(part 1 of 4)
# Autodesk Inventor assembly: FRC Fixed Field 2018_sldasm
Saved by Autodesk Inventor 2016 SP2 (Build 200236200, 236)
## iProperties
Created: 2018-01-13
Part Number: FRC Fixed Field 2018_sldasm
Document SubType Name: Assembly
Designer: CAD
Author: CAD
## Documents named in this file (943)
- C:\Users\CAD\Documents\GitHub\FIRST-ROBOTICS-2018-5436-CAD\Field\FIRST Power Up Field CAD\FRC Fixed Field 2018_sldasm.iam
- C:\Users\CAD\Documents\GitHub\FIRST-ROBOTICS-2018-5436-CAD\Field\FIRST Power Up Field CAD\Body_525_sldprt.ipt
- C:\Users\CAD\Documents\GitHub\FIRST-ROBOTICS-2018-5436-CAD\Field\FIRST Power Up Field CAD\Body_526_sldprt.ipt
- C:\Users\CAD\Documents\GitHub\FIRST-ROBOTICS-2018-5436-CAD\Field\FIRST Power Up Field CAD\Body_527_sldprt.ipt
- C:\Users\CAD\Documents\GitHub\FIRST-ROBOTICS-2018-5436-CAD\Field\FIRST Power Up Field CAD\Body_528_sldprt.ipt
- C:\Users\CAD\Documents\GitHub\FIRST-ROBOTICS-2018-5436-CAD\Field\FIRST Power Up Field CAD\Body_529_sldprt.ipt
- C:\Users\CAD\Documents\GitHub\FIRST-ROBOTICS-2018-5436-CAD\Field\FIRST Power Up Field CAD\Body_530_sldprt.ipt
- C:\Users\CAD\Documents\GitHub\FIRST-ROBOTICS-2018-5436-CAD\Field\FIRST Power Up Field CAD\Body_531_sldprt.ipt
- C:\Users\CAD\Documents\GitHub\FIRST-ROBOTICS-2018-5436-CAD\Field\FIRST Power Up Field CAD\Body_532_sldprt.ipt
- C:\Users\CAD\Documents\GitHub\FIRST-ROBOTICS-2018-5436-CAD\Field\FIRST Power Up Field CAD\Body_533_sldprt.ipt
- C:\Users\CAD\Documents\GitHub\FIRST-ROBOTICS-2018-5436-CAD\Field\FIRST Power Up Field CAD\Body_534_sldprt.ipt
- C:\Users\CAD\Documents\GitHub\FIRST-ROBOTICS-2018-5436-CAD\Field\FIRST Power Up Field CAD\Body_535_sldprt.ipt
- C:\Users\CAD\Documents\GitHub\FIRST-ROBOTICS-2018-5436-CAD\Field\FIRST Power Up Field CAD\Body_536_sldprt.ipt
- C:\Users\CAD\Documents\GitHub\FIRST-ROBOTICS-2018-5436-CAD\Field\FIRST Power Up Field CAD\Body_537_sldprt.ipt
- C:\Users\CAD\Documents\GitHub\FIRST-ROBOTICS-2018-5436-CAD\Field\FIRST Power Up Field CAD\Body_538_sldprt.ipt
- C:\Users\CAD\Documents\GitHub\FIRST-ROBOTICS-2018-5436-CAD\Field\FIRST Power Up Field CAD\Body_539_sldprt.ipt
- C:\Users\CAD\Documents\GitHub\FIRST-ROBOTICS-2018-5436-CAD\Field\FIRST Power Up Field CAD\Body_540_sldprt.ipt
- C:\Users\CAD\Documents\GitHub\FIRST-ROBOTICS-2018-5436-CAD\Field\FIRST Power Up Field CAD\Body_541_sldprt.ipt
- C:\Users\CAD\Documents\GitHub\FIRST-ROBOTICS-2018-5436-CAD\Field\FIRST Power Up Field CAD\Body_542_sldprt.ipt
- C:\Users\CAD\Documents\GitHub\FIRST-ROBOTICS-2018-5436-CAD\Field\FIRST Power Up Field CAD\Body_543_sldprt.ipt
- C:\Users\CAD\Documents\GitHub\FIRST-ROBOTICS-2018-5436-CAD\Field\FIRST Power Up Field CAD\Body_544_sldprt.ipt
- C:\Users\CAD\Documents\GitHub\FIRST-ROBOTICS-2018-5436-CAD\Field\FIRST Power Up Field CAD\Body_545_sldprt.ipt
- C:\Users\CAD\Documents\GitHub\FIRST-ROBOTICS-2018-5436-CAD\Field\FIRST Power Up Field CAD\Body_546_sldprt.ipt
- C:\Users\CAD\Documents\GitHub\FIRST-ROBOTICS-2018-5436-CAD\Field\FIRST Power Up Field CAD\Body_547_sldprt.ipt
- C:\Users\CAD\Documents\GitHub\FIRST-ROBOTICS-2018-5436-CAD\Field\FIRST Power Up Field CAD\Body_548_sldprt.ipt
- C:\Users\CAD\Documents\GitHub\FIRST-ROBOTICS-2018-5436-CAD\Field\FIRST Power Up Field CAD\Body_549_sldprt.ipt
- C:\Users\CAD\Documents\GitHub\FIRST-ROBOTICS-2018-5436-CAD\Field\FIRST Power Up Field CAD\Body_550_sldprt.ipt
- C:\Users\CAD\Documents\GitHub\FIRST-ROBOTICS-2018-5436-CAD\Field\FIRST Power Up Field CAD\Body_551_sldprt.ipt
- C:\Users\CAD\Documents\GitHub\FIRST-ROBOTICS-2018-5436-CAD\Field\FIRST Power Up Field CAD\Body_552_sldprt.ipt
- C:\Users\CAD\Documents\GitHub\FIRST-ROBOTICS-2018-5436-CAD\Field\FIRST Power Up Field CAD\Body_553_sldprt.ipt
- C:\Users\CAD\Documents\GitHub\FIRST-ROBOTICS-2018-5436-CAD\Field\FIRST Power Up Field CAD\Body_554_sldprt.ipt
- C:\Users\CAD\Documents\GitHub\FIRST-ROBOTICS-2018-5436-CAD\Field\FIRST Power Up Field CAD\Body_555_sldprt.ipt
- C:\Users\CAD\Documents\GitHub\FIRST-ROBOTICS-2018-5436-CAD\Field\FIRST Power Up Field CAD\Body_556_sldprt.ipt
- C:\Users\CAD\Documents\GitHub\FIRST-ROBOTICS-2018-5436-CAD\Field\FIRST Power Up Field CAD\Body_557_sldprt.ipt
- C:\Users\CAD\Documents\GitHub\FIRST-ROBOTICS-2018-5436-CAD\Field\FIRST Power Up Field CAD\Body_558_sldprt.ipt
- C:\Users\CAD\Documents\GitHub\FIRST-ROBOTICS-2018-5436-CAD\Field\FIRST Power Up Field CAD\Body_559_sldprt.ipt
- C:\Users\CAD\Documents\GitHub\FIRST-ROBOTICS-2018-5436-CAD\Field\FIRST Power Up Field CAD\Body_560_sldprt.ipt
- C:\Users\CAD\Documents\GitHub\FIRST-ROBOTICS-2018-5436-CAD\Field\FIRST Power Up Field CAD\Body_561_sldprt.ipt
- C:\Users\CAD\Documents\GitHub\FIRST-ROBOTICS-2018-5436-CAD\Field\FIRST Power Up Field CAD\Body_562_sldprt.ipt
- C:\Users\CAD\Documents\GitHub\FIRST-ROBOTICS-2018-5436-CAD\Field\FIRST Power Up Field CAD\Body_563_sldprt.ipt
- C:\Users\CAD\Documents\GitHub\FIRST-ROBOTICS-2018-5436-CAD\Field\FIRST Power Up Field CAD\Body_564_sldprt.ipt
- C:\Users\CAD\Documents\GitHub\FIRST-ROBOTICS-2018-5436-CAD\Field\FIRST Power Up Field CAD\Body_565_sldprt.ipt
- C:\Users\CAD\Documents\GitHub\FIRST-ROBOTICS-2018-5436-CAD\Field\FIRST Power Up Field CAD\Body_566_sldprt.ipt
- C:\Users\CAD\Documents\GitHub\FIRST-ROBOTICS-2018-5436-CAD\Field\FIRST Power Up Field CAD\Body_567_sldprt.ipt
- C:\Users\CAD\Documents\GitHub\FIRST-ROBOTICS-2018-5436-CAD\Field\FIRST Power Up Field CAD\Body_568_sldprt.ipt
- C:\Users\CAD\Documents\GitHub\FIRST-ROBOTICS-2018-5436-CAD\Field\FIRST Power Up Field CAD\Body_569_sldprt.ipt
- C:\Users\CAD\Documents\GitHub\FIRST-ROBOTICS-2018-5436-CAD\Field\FIRST Power Up Field CAD\Body_570_sldprt.ipt
- C:\Users\CAD\Documents\GitHub\FIRST-ROBOTICS-2018-5436-CAD\Field\FIRST Power Up Field CAD\Body_571_sldprt.ipt
- C:\Users\CAD\Documents\GitHub\FIRST-ROBOTICS-2018-5436-CAD\Field\FIRST Power Up Field CAD\Body_572_sldprt.ipt
- C:\Users\CAD\Documents\GitHub\FIRST-ROBOTICS-2018-5436-CAD\Field\FIRST Power Up Field CAD\Body_573_sldprt.ipt
- C:\Users\CAD\Documents\GitHub\FIRST-ROBOTICS-2018-5436-CAD\Field\FIRST Power Up Field CAD\Body_574_sldprt.ipt
- C:\Users\CAD\Documents\GitHub\FIRST-ROBOTICS-2018-5436-CAD\Field\FIRST Power Up Field CAD\Body_575_sldprt.ipt
- C:\Users\CAD\Documents\GitHub\FIRST-ROBOTICS-2018-5436-CAD\Field\FIRST Power Up Field CAD\Body_576_sldprt.ipt
- C:\Users\CAD\Documents\GitHub\FIRST-ROBOTICS-2018-5436-CAD\Field\FIRST Power Up Field CAD\Body_577_sldprt.ipt
- C:\Users\CAD\Documents\GitHub\FIRST-ROBOTICS-2018-5436-CAD\Field\FIRST Power Up Field CAD\Body_578_sldprt.ipt
- C:\Users\CAD\Documents\GitHub\FIRST-ROBOTICS-2018-5436-CAD\Field\FIRST Power Up Field CAD\Body_579_sldprt.ipt
- C:\Users\CAD\Documents\GitHub\FIRST-ROBOTICS-2018-5436-CAD\Field\FIRST Power Up Field CAD\Body_580_sldprt.ipt
- C:\Users\CAD\Documents\GitHub\FIRST-ROBOTICS-2018-5436-CAD\Field\FIRST Power Up Field CAD\Body_581_sldprt.ipt
- C:\Users\CAD\Documents\GitHub\FIRST-ROBOTICS-2018-5436-CAD\Field\FIRST Power Up Field CAD\Body_582_sldprt.ipt
- C:\Users\CAD\Documents\GitHub\FIRST-ROBOTICS-2018-5436-CAD\Field\FIRST Power Up Field CAD\Body_583_sldprt.ipt
- C:\Users\CAD\Documents\GitHub\FIRST-ROBOTICS-2018-5436-CAD\Field\FIRST Power Up Field CAD\Body_584_sldprt.ipt
- C:\Users\CAD\Documents\GitHub\FIRST-ROBOTICS-2018-5436-CAD\Field\FIRST Power Up Field CAD\Body_585_sldprt.ipt
- C:\Users\CAD\Documents\GitHub\FIRST-ROBOTICS-2018-5436-CAD\Field\FIRST Power Up Field CAD\Body_586_sldprt.ipt
- C:\Users\CAD\Documents\GitHub\FIRST-ROBOTICS-2018-5436-CAD\Field\FIRST Power Up Field CAD\Body_587_sldprt.ipt
- C:\Users\CAD\Documents\GitHub\FIRST-ROBOTICS-2018-5436-CAD\Field\FIRST Power Up Field CAD\Body_588_sldprt.ipt
- C:\Users\CAD\Documents\GitHub\FIRST-ROBOTICS-2018-5436-CAD\Field\FIRST Power Up Field CAD\Body_589_sldprt.ipt
- C:\Users\CAD\Documents\GitHub\FIRST-ROBOTICS-2018-5436-CAD\Field\FIRST Power Up Field CAD\Body_590_sldprt.ipt
- C:\Users\CAD\Documents\GitHub\FIRST-ROBOTICS-2018-5436-CAD\Field\FIRST Power Up Field CAD\Body_591_sldprt.ipt
- C:\Users\CAD\Documents\GitHub\FIRST-ROBOTICS-2018-5436-CAD\Field\FIRST Power Up Field CAD\Body_592_sldprt.ipt
- C:\Users\CAD\Documents\GitHub\FIRST-ROBOTICS-2018-5436-CAD\Field\FIRST Power Up Field CAD\Body_593_sldprt.ipt
- C:\Users\CAD\Documents\GitHub\FIRST-ROBOTICS-2018-5436-CAD\Field\FIRST Power Up Field CAD\Body_594_sldprt.ipt
- C:\Users\CAD\Documents\GitHub\FIRST-ROBOTICS-2018-5436-CAD\Field\FIRST Power Up Field CAD\Body_595_sldprt.ipt
- C:\Users\CAD\Documents\GitHub\FIRST-ROBOTICS-2018-5436-CAD\Field\FIRST Power Up Field CAD\Body_596_sldprt.ipt
- C:\Users\CAD\Documents\GitHub\FIRST-ROBOTICS-2018-5436-CAD\Field\FIRST Power Up Field CAD\Body_597_sldprt.ipt
- C:\Users\CAD\Documents\GitHub\FIRST-ROBOTICS-2018-5436-CAD\Field\FIRST Power Up Field CAD\Body_598_sldprt.ipt
- C:\Users\CAD\Documents\GitHub\FIRST-ROBOTICS-2018-5436-CAD\Field\FIRST Power Up Field CAD\Body_599_sldprt.ipt
- C:\Users\CAD\Documents\GitHub\FIRST-ROBOTICS-2018-5436-CAD\Field\FIRST Power Up Field CAD\Body_600_sldprt.ipt
- C:\Users\CAD\Documents\GitHub\FIRST-ROBOTICS-2018-5436-CAD\Field\FIRST Power Up Field CAD\Body_601_sldprt.ipt
- C:\Users\CAD\Documents\GitHub\FIRST-ROBOTICS-2018-5436-CAD\Field\FIRST Power Up Field CAD\Body_602_sldprt.ipt
- C:\Users\CAD\Documents\GitHub\FIRST-ROBOTICS-2018-5436-CAD\Field\FIRST Power Up Field CAD\Body_603_sldprt.ipt
- C:\Users\CAD\Documents\GitHub\FIRST-ROBOTICS-2018-5436-CAD\Field\FIRST Power Up Field CAD\Body_604_sldprt.ipt
- C:\Users\CAD\Documents\GitHub\FIRST-ROBOTICS-2018-5436-CAD\Field\FIRST Power Up Field CAD\Body_605_sldprt.ipt
- C:\Users\CAD\Documents\GitHub\FIRST-ROBOTICS-2018-5436-CAD\Field\FIRST Power Up Field CAD\Body_606_sldprt.ipt
- C:\Users\CAD\Documents\GitHub\FIRST-ROBOTICS-2018-5436-CAD\Field\FIRST Power Up Field CAD\Body_607_sldprt.ipt
- C:\Users\CAD\Documents\GitHub\FIRST-ROBOTICS-2018-5436-CAD\Field\FIRST Power Up Field CAD\Body_608_sldprt.ipt
- C:\Users\CAD\Documents\GitHub\FIRST-ROBOTICS-2018-5436-CAD\Field\FIRST Power Up Field CAD\Body_609_sldprt.ipt
- C:\Users\CAD\Documents\GitHub\FIRST-ROBOTICS-2018-5436-CAD\Field\FIRST Power Up Field CAD\Body_610_sldprt.ipt
- C:\Users\CAD\Documents\GitHub\FIRST-ROBOTICS-2018-5436-CAD\Field\FIRST Power Up Field CAD\Body_611_sldprt.ipt
- C:\Users\CAD\Documents\GitHub\FIRST-ROBOTICS-2018-5436-CAD\Field\FIRST Power Up Field CAD\Body_612_sldprt.ipt
- C:\Users\CAD\Documents\GitHub\FIRST-ROBOTICS-2018-5436-CAD\Field\FIRST Power Up Field CAD\Body_613_sldprt.ipt
- C:\Users\CAD\Documents\GitHub\FIRST-ROBOTICS-2018-5436-CAD\Field\FIRST Power Up Field CAD\Body_614_sldprt.ipt
- C:\Users\CAD\Documents\GitHub\FIRST-ROBOTICS-2018-5436-CAD\Field\FIRST Power Up Field CAD\Body_615_sldprt.ipt
- C:\Users\CAD\Documents\GitHub\FIRST-ROBOTICS-2018-5436-CAD\Field\FIRST Power Up Field CAD\Body_616_sldprt.ipt
- C:\Users\CAD\Documents\GitHub\FIRST-ROBOTICS-2018-5436-CAD\Field\FIRST Power Up Field CAD\Body_617_sldprt.ipt
- C:\Users\CAD\Documents\GitHub\FIRST-ROBOTICS-2018-5436-CAD\Field\FIRST Power Up Field CAD\Body_618_sldprt.ipt
- C:\Users\CAD\Documents\GitHub\FIRST-ROBOTICS-2018-5436-CAD\Field\FIRST Power Up Field CAD\Body_619_sldprt.ipt
- C:\Users\CAD\Documents\GitHub\FIRST-ROBOTICS-2018-5436-CAD\Field\FIRST Power Up Field CAD\Body_620_sldprt.ipt
- C:\Users\CAD\Documents\GitHub\FIRST-ROBOTICS-2018-5436-CAD\Field\FIRST Power Up Field CAD\Body_621_sldprt.ipt
- C:\Users\CAD\Documents\GitHub\FIRST-ROBOTICS-2018-5436-CAD\Field\FIRST Power Up Field CAD\Body_622_sldprt.ipt
- C:\Users\CAD\Documents\GitHub\FIRST-ROBOTICS-2018-5436-CAD\Field\FIRST Power Up Field CAD\Body_623_sldprt.ipt
- C:\Users\CAD\Documents\GitHub\FIRST-ROBOTICS-2018-5436-CAD\Field\FIRST Power Up Field CAD\Body_624_sldprt.ipt
- C:\Users\CAD\Documents\GitHub\FIRST-ROBOTICS-2018-5436-CAD\Field\FIRST Power Up Field CAD\Body_625_sldprt.ipt
- C:\Users\CAD\Documents\GitHub\FIRST-ROBOTICS-2018-5436-CAD\Field\FIRST Power Up Field CAD\Body_626_sldprt.ipt
- C:\Users\CAD\Documents\GitHub\FIRST-ROBOTICS-2018-5436-CAD\Field\FIRST Power Up Field CAD\Body_627_sldprt.ipt
- C:\Users\CAD\Documents\GitHub\FIRST-ROBOTICS-2018-5436-CAD\Field\FIRST Power Up Field CAD\Body_628_sldprt.ipt
- C:\Users\CAD\Documents\GitHub\FIRST-ROBOTICS-2018-5436-CAD\Field\FIRST Power Up Field CAD\Body_629_sldprt.ipt
- C:\Users\CAD\Documents\GitHub\FIRST-ROBOTICS-2018-5436-CAD\Field\FIRST Power Up Field CAD\Body_630_sldprt.ipt
- C:\Users\CAD\Documents\GitHub\FIRST-ROBOTICS-2018-5436-CAD\Field\FIRST Power Up Field CAD\Body_631_sldprt.ipt
- C:\Users\CAD\Documents\GitHub\FIRST-ROBOTICS-2018-5436-CAD\Field\FIRST Power Up Field CAD\Body_632_sldprt.ipt
- C:\Users\CAD\Documents\GitHub\FIRST-ROBOTICS-2018-5436-CAD\Field\FIRST Power Up Field CAD\Body_633_sldprt.ipt
- C:\Users\CAD\Documents\GitHub\FIRST-ROBOTICS-2018-5436-CAD\Field\FIRST Power Up Field CAD\Body_634_sldprt.ipt
- C:\Users\CAD\Documents\GitHub\FIRST-ROBOTICS-2018-5436-CAD\Field\FIRST Power Up Field CAD\Body_635_sldprt.ipt
- C:\Users\CAD\Documents\GitHub\FIRST-ROBOTICS-2018-5436-CAD\Field\FIRST Power Up Field CAD\Body_636_sldprt.ipt
- C:\Users\CAD\Documents\GitHub\FIRST-ROBOTICS-2018-5436-CAD\Field\FIRST Power Up Field CAD\Body_637_sldprt.ipt
- C:\Users\CAD\Documents\GitHub\FIRST-ROBOTICS-2018-5436-CAD\Field\FIRST Power Up Field CAD\Body_638_sldprt.ipt
- C:\Users\CAD\Documents\GitHub\FIRST-ROBOTICS-2018-5436-CAD\Field\FIRST Power Up Field CAD\Body_639_sldprt.ipt
- C:\Users\CAD\Documents\GitHub\FIRST-ROBOTICS-2018-5436-CAD\Field\FIRST Power Up Field CAD\Body_640_sldprt.ipt
- C:\Users\CAD\Documents\GitHub\FIRST-ROBOTICS-2018-5436-CAD\Field\FIRST Power Up Field CAD\Body_641_sldprt.ipt
- C:\Users\CAD\Documents\GitHub\FIRST-ROBOTICS-2018-5436-CAD\Field\FIRST Power Up Field CAD\Body_642_sldprt.ipt
- C:\Users\CAD\Documents\GitHub\FIRST-ROBOTICS-2018-5436-CAD\Field\FIRST Power Up Field CAD\Body_643_sldprt.ipt
- C:\Users\CAD\Documents\GitHub\FIRST-ROBOTICS-2018-5436-CAD\Field\FIRST Power Up Field CAD\Body_644_sldprt.ipt
- C:\Users\CAD\Documents\GitHub\FIRST-ROBOTICS-2018-5436-CAD\Field\FIRST Power Up Field CAD\Body_645_sldprt.ipt
- C:\Users\CAD\Documents\GitHub\FIRST-ROBOTICS-2018-5436-CAD\Field\FIRST Power Up Field CAD\Body_646_sldprt.ipt
- C:\Users\CAD\Documents\GitHub\FIRST-ROBOTICS-2018-5436-CAD\Field\FIRST Power Up Field CAD\Body_647_sldprt.ipt
- C:\Users\CAD\Documents\GitHub\FIRST-ROBOTICS-2018-5436-CAD\Field\FIRST Power Up Field CAD\Body_648_sldprt.ipt
- C:\Users\CAD\Documents\GitHub\FIRST-ROBOTICS-2018-5436-CAD\Field\FIRST Power Up Field CAD\Body_649_sldprt.ipt
- C:\Users\CAD\Documents\GitHub\FIRST-ROBOTICS-2018-5436-CAD\Field\FIRST Power Up Field CAD\Body_650_sldprt.ipt
- C:\Users\CAD\Documents\GitHub\FIRST-ROBOTICS-2018-5436-CAD\Field\FIRST Power Up Field CAD\Body_651_sldprt.ipt
- C:\Users\CAD\Documents\GitHub\FIRST-ROBOTICS-2018-5436-CAD\Field\FIRST Power Up Field CAD\Body_652_sldprt.ipt
- C:\Users\CAD\Documents\GitHub\FIRST-ROBOTICS-2018-5436-CAD\Field\FIRST Power Up Field CAD\Body_653_sldprt.ipt
- C:\Users\CAD\Documents\GitHub\FIRST-ROBOTICS-2018-5436-CAD\Field\FIRST Power Up Field CAD\Body_654_sldprt.ipt
- C:\Users\CAD\Documents\GitHub\FIRST-ROBOTICS-2018-5436-CAD\Field\FIRST Power Up Field CAD\Body_655_sldprt.ipt
- C:\Users\CAD\Documents\GitHub\FIRST-ROBOTICS-2018-5436-CAD\Field\FIRST Power Up Field CAD\Body_656_sldprt.ipt
- C:\Users\CAD\Documents\GitHub\FIRST-ROBOTICS-2018-5436-CAD\Field\FIRST Power Up Field CAD\Body_657_sldprt.ipt
- C:\Users\CAD\Documents\GitHub\FIRST-ROBOTICS-2018-5436-CAD\Field\FIRST Power Up Field CAD\Body_658_sldprt.ipt
- C:\Users\CAD\Documents\GitHub\FIRST-ROBOTICS-2018-5436-CAD\Field\FIRST Power Up Field CAD\Body_659_sldprt.ipt
- C:\Users\CAD\Documents\GitHub\FIRST-ROBOTICS-2018-5436-CAD\Field\FIRST Power Up Field CAD\Body_660_sldprt.ipt
- C:\Users\CAD\Documents\GitHub\FIRST-ROBOTICS-2018-5436-CAD\Field\FIRST Power Up Field CAD\Body_661_sldprt.ipt
- C:\Users\CAD\Documents\GitHub\FIRST-ROBOTICS-2018-5436-CAD\Field\FIRST Power Up Field CAD\Body_662_sldprt.ipt
- C:\Users\CAD\Documents\GitHub\FIRST-ROBOTICS-2018-5436-CAD\Field\FIRST Power Up Field CAD\Body_663_sldprt.ipt
- C:\Users\CAD\Documents\GitHub\FIRST-ROBOTICS-2018-5436-CAD\Field\FIRST Power Up Field CAD\Body_664_sldprt.ipt
- C:\Users\CAD\Documents\GitHub\FIRST-ROBOTICS-2018-5436-CAD\Field\FIRST Power Up Field CAD\Body_665_sldprt.ipt
- C:\Users\CAD\Documents\GitHub\FIRST-ROBOTICS-2018-5436-CAD\Field\FIRST Power Up Field CAD\Body_666_sldprt.ipt
- C:\Users\CAD\Documents\GitHub\FIRST-ROBOTICS-2018-5436-CAD\Field\FIRST Power Up Field CAD\Body_667_sldprt.ipt
- C:\Users\CAD\Documents\GitHub\FIRST-ROBOTICS-2018-5436-CAD\Field\FIRST Power Up Field CAD\Body_668_sldprt.ipt
- C:\Users\CAD\Documents\GitHub\FIRST-ROBOTICS-2018-5436-CAD\Field\FIRST Power Up Field CAD\Body_669_sldprt.ipt
- C:\Users\CAD\Documents\GitHub\FIRST-ROBOTICS-2018-5436-CAD\Field\FIRST Power Up Field CAD\Body_670_sldprt.ipt
- C:\Users\CAD\Documents\GitHub\FIRST-ROBOTICS-2018-5436-CAD\Field\FIRST Power Up Field CAD\Body_671_sldprt.ipt
- C:\Users\CAD\Documents\GitHub\FIRST-ROBOTICS-2018-5436-CAD\Field\FIRST Power Up Field CAD\Body_672_sldprt.ipt
- C:\Users\CAD\Documents\GitHub\FIRST-ROBOTICS-2018-5436-CAD\Field\FIRST Power Up Field CAD\Body_673_sldprt.ipt
- C:\Users\CAD\Documents\GitHub\FIRST-ROBOTICS-2018-5436-CAD\Field\FIRST Power Up Field CAD\Body_674_sldprt.ipt
- C:\Users\CAD\Documents\GitHub\FIRST-ROBOTICS-2018-5436-CAD\Field\FIRST Power Up Field CAD\Body_675_sldprt.ipt
- C:\Users\CAD\Documents\GitHub\FIRST-ROBOTICS-2018-5436-CAD\Field\FIRST Power Up Field CAD\Body_676_sldprt.ipt
- C:\Users\CAD\Documents\GitHub\FIRST-ROBOTICS-2018-5436-CAD\Field\FIRST Power Up Field CAD\Body_677_sldprt.ipt
- C:\Users\CAD\Documents\GitHub\FIRST-ROBOTICS-2018-5436-CAD\Field\FIRST Power Up Field CAD\Body_678_sldprt.ipt
- C:\Users\CAD\Documents\GitHub\FIRST-ROBOTICS-2018-5436-CAD\Field\FIRST Power Up Field CAD\Body_679_sldprt.ipt
- C:\Users\CAD\Documents\GitHub\FIRST-ROBOTICS-2018-5436-CAD\Field\FIRST Power Up Field CAD\Body_680_sldprt.ipt
- C:\Users\CAD\Documents\GitHub\FIRST-ROBOTICS-2018-5436-CAD\Field\FIRST Power Up Field CAD\Body_681_sldprt.ipt
- C:\Users\CAD\Documents\GitHub\FIRST-ROBOTICS-2018-5436-CAD\Field\FIRST Power Up Field CAD\Body_682_sldprt.ipt
- C:\Users\CAD\Documents\GitHub\FIRST-ROBOTICS-2018-5436-CAD\Field\FIRST Power Up Field CAD\Body_683_sldprt.ipt
- C:\Users\CAD\Documents\GitHub\FIRST-ROBOTICS-2018-5436-CAD\Field\FIRST Power Up Field CAD\Body_684_sldprt.ipt
- C:\Users\CAD\Documents\GitHub\FIRST-ROBOTICS-2018-5436-CAD\Field\FIRST Power Up Field CAD\Body_685_sldprt.ipt
- C:\Users\CAD\Documents\GitHub\FIRST-ROBOTICS-2018-5436-CAD\Field\FIRST Power Up Field CAD\Body_686_sldprt.ipt
- C:\Users\CAD\Documents\GitHub\FIRST-ROBOTICS-2018-5436-CAD\Field\FIRST Power Up Field CAD\Body_687_sldprt.ipt
- C:\Users\CAD\Documents\GitHub\FIRST-ROBOTICS-2018-5436-CAD\Field\FIRST Power Up Field CAD\Body_688_sldprt.ipt
- C:\Users\CAD\Documents\GitHub\FIRST-ROBOTICS-2018-5436-CAD\Field\FIRST Power Up Field CAD\Body_689_sldprt.ipt
- C:\Users\CAD\Documents\GitHub\FIRST-ROBOTICS-2018-5436-CAD\Field\FIRST Power Up Field CAD\Body_690_sldprt.ipt
- C:\Users\CAD\Documents\GitHub\FIRST-ROBOTICS-2018-5436-CAD\Field\FIRST Power Up Field CAD\Body_691_sldprt.ipt
- C:\Users\CAD\Documents\GitHub\FIRST-ROBOTICS-2018-5436-CAD\Field\FIRST Power Up Field CAD\Body_692_sldprt.ipt
- C:\Users\CAD\Documents\GitHub\FIRST-ROBOTICS-2018-5436-CAD\Field\FIRST Power Up Field CAD\Body_693_sldprt.ipt
- C:\Users\CAD\Documents\GitHub\FIRST-ROBOTICS-2018-5436-CAD\Field\FIRST Power Up Field CAD\Body_694_sldprt.ipt
- C:\Users\CAD\Documents\GitHub\FIRST-ROBOTICS-2018-5436-CAD\Field\FIRST Power Up Field CAD\Body_695_sldprt.ipt
- C:\Users\CAD\Documents\GitHub\FIRST-ROBOTICS-2018-5436-CAD\Field\FIRST Power Up Field CAD\Body_696_sldprt.ipt
- C:\Users\CAD\Documents\GitHub\FIRST-ROBOTICS-2018-5436-CAD\Field\FIRST Power Up Field CAD\Body_697_sldprt.ipt
- C:\Users\CAD\Documents\GitHub\FIRST-ROBOTICS-2018-5436-CAD\Field\FIRST Power Up Field CAD\Body_698_sldprt.ipt
- C:\Users\CAD\Documents\GitHub\FIRST-ROBOTICS-2018-5436-CAD\Field\FIRST Power Up Field CAD\Body_699_sldprt.ipt
- C:\Users\CAD\Documents\GitHub\FIRST-ROBOTICS-2018-5436-CAD\Field\FIRST Power Up Field CAD\Body_700_sldprt.ipt
- C:\Users\CAD\Documents\GitHub\FIRST-ROBOTICS-2018-5436-CAD\Field\FIRST Power Up Field CAD\Body_701_sldprt.ipt
- C:\Users\CAD\Documents\GitHub\FIRST-ROBOTICS-2018-5436-CAD\Field\FIRST Power Up Field CAD\Body_702_sldprt.ipt
- C:\Users\CAD\Documents\GitHub\FIRST-ROBOTICS-2018-5436-CAD\Field\FIRST Power Up Field CAD\Body_703_sldprt.ipt
- C:\Users\CAD\Documents\GitHub\FIRST-ROBOTICS-2018-5436-CAD\Field\FIRST Power Up Field CAD\Body_704_sldprt.ipt
- C:\Users\CAD\Documents\GitHub\FIRST-ROBOTICS-2018-5436-CAD\Field\FIRST Power Up Field CAD\Body_705_sldprt.ipt
- C:\Users\CAD\Documents\GitHub\FIRST-ROBOTICS-2018-5436-CAD\Field\FIRST Power Up Field CAD\Body_706_sldprt.ipt
- C:\Users\CAD\Documents\GitHub\FIRST-ROBOTICS-2018-5436-CAD\Field\FIRST Power Up Field CAD\Body_707_sldprt.ipt
- C:\Users\CAD\Documents\GitHub\FIRST-ROBOTICS-2018-5436-CAD\Field\FIRST Power Up Field CAD\Body_708_sldprt.ipt
- C:\Users\CAD\Documents\GitHub\FIRST-ROBOTICS-2018-5436-CAD\Field\FIRST Power Up Field CAD\Body_709_sldprt.ipt
- C:\Users\CAD\Documents\GitHub\FIRST-ROBOTICS-2018-5436-CAD\Field\FIRST Power Up Field CAD\Body_710_sldprt.ipt
- C:\Users\CAD\Documents\GitHub\FIRST-ROBOTICS-2018-5436-CAD\Field\FIRST Power Up Field CAD\Body_711_sldprt.ipt
- C:\Users\CAD\Documents\GitHub\FIRST-ROBOTICS-2018-5436-CAD\Field\FIRST Power Up Field CAD\Body_712_sldprt.ipt
- C:\Users\CAD\Documents\GitHub\FIRST-ROBOTICS-2018-5436-CAD\Field\FIRST Power Up Field CAD\Body_713_sldprt.ipt
- C:\Users\CAD\Documents\GitHub\FIRST-ROBOTICS-2018-5436-CAD\Field\FIRST Power Up Field CAD\Body_714_sldprt.ipt
- C:\Users\CAD\Documents\GitHub\FIRST-ROBOTICS-2018-5436-CAD\Field\FIRST Power Up Field CAD\Body_715_sldprt.ipt
- C:\Users\CAD\Documents\GitHub\FIRST-ROBOTICS-2018-5436-CAD\Field\FIRST Power Up Field CAD\Body_716_sldprt.ipt
- C:\Users\CAD\Documents\GitHub\FIRST-ROBOTICS-2018-5436-CAD\Field\FIRST Power Up Field CAD\Body_717_sldprt.ipt
- C:\Users\CAD\Documents\GitHub\FIRST-ROBOTICS-2018-5436-CAD\Field\FIRST Power Up Field CAD\Body_718_sldprt.ipt
- C:\Users\CAD\Documents\GitHub\FIRST-ROBOTICS-2018-5436-CAD\Field\FIRST Power Up Field CAD\Body_719_sldprt.ipt
- C:\Users\CAD\Documents\GitHub\FIRST-ROBOTICS-2018-5436-CAD\Field\FIRST Power Up Field CAD\Body_720_sldprt.ipt
- C:\Users\CAD\Documents\GitHub\FIRST-ROBOTICS-2018-5436-CAD\Field\FIRST Power Up Field CAD\Body_721_sldprt.ipt
- C:\Users\CAD\Documents\GitHub\FIRST-ROBOTICS-2018-5436-CAD\Field\FIRST Power Up Field CAD\Body_722_sldprt.ipt
- C:\Users\CAD\Documents\GitHub\FIRST-ROBOTICS-2018-5436-CAD\Field\FIRST Power Up Field CAD\Body_723_sldprt.ipt
- C:\Users\CAD\Documents\GitHub\FIRST-ROBOTICS-2018-5436-CAD\Field\FIRST Power Up Field CAD\Body_724_sldprt.ipt
- C:\Users\CAD\Documents\GitHub\FIRST-ROBOTICS-2018-5436-CAD\Field\FIRST Power Up Field CAD\Body_725_sldprt.ipt
- C:\Users\CAD\Documents\GitHub\FIRST-ROBOTICS-2018-5436-CAD\Field\FIRST Power Up Field CAD\Body_726_sldprt.ipt
- C:\Users\CAD\Documents\GitHub\FIRST-ROBOTICS-2018-5436-CAD\Field\FIRST Power Up Field CAD\Body_727_sldprt.ipt
- C:\Users\CAD\Documents\GitHub\FIRST-ROBOTICS-2018-5436-CAD\Field\FIRST Power Up Field CAD\Body_728_sldprt.ipt
- C:\Users\CAD\Documents\GitHub\FIRST-ROBOTICS-2018-5436-CAD\Field\FIRST Power Up Field CAD\Body_729_sldprt.ipt
- C:\Users\CAD\Documents\GitHub\FIRST-ROBOTICS-2018-5436-CAD\Field\FIRST Power Up Field CAD\Body_730_sldprt.ipt
- C:\Users\CAD\Documents\GitHub\FIRST-ROBOTICS-2018-5436-CAD\Field\FIRST Power Up Field CAD\Body_731_sldprt.ipt
- C:\Users\CAD\Documents\GitHub\FIRST-ROBOTICS-2018-5436-CAD\Field\FIRST Power Up Field CAD\Body_732_sldprt.ipt
- C:\Users\CAD\Documents\GitHub\FIRST-ROBOTICS-2018-5436-CAD\Field\FIRST Power Up Field CAD\Body_733_sldprt.ipt
- C:\Users\CAD\Documents\GitHub\FIRST-ROBOTICS-2018-5436-CAD\Field\FIRST Power Up Field CAD\Body_734_sldprt.ipt
- C:\Users\CAD\Documents\GitHub\FIRST-ROBOTICS-2018-5436-CAD\Field\FIRST Power Up Field CAD\Body_735_sldprt.ipt
- C:\Users\CAD\Documents\GitHub\FIRST-ROBOTICS-2018-5436-CAD\Field\FIRST Power Up Field CAD\Body_736_sldprt.ipt
- C:\Users\CAD\Documents\GitHub\FIRST-ROBOTICS-2018-5436-CAD\Field\FIRST Power Up Field CAD\Body_737_sldprt.ipt
- C:\Users\CAD\Documents\GitHub\FIRST-ROBOTICS-2018-5436-CAD\Field\FIRST Power Up Field CAD\Body_738_sldprt.ipt
- C:\Users\CAD\Documents\GitHub\FIRST-ROBOTICS-2018-5436-CAD\Field\FIRST Power Up Field CAD\Body_739_sldprt.ipt
- C:\Users\CAD\Documents\GitHub\FIRST-ROBOTICS-2018-5436-CAD\Field\FIRST Power Up Field CAD\Body_740_sldprt.ipt
- C:\Users\CAD\Documents\GitHub\FIRST-ROBOTICS-2018-5436-CAD\Field\FIRST Power Up Field CAD\Body_741_sldprt.ipt
- C:\Users\CAD\Documents\GitHub\FIRST-ROBOTICS-2018-5436-CAD\Field\FIRST Power Up Field CAD\Body_742_sldprt.ipt
- C:\Users\CAD\Documents\GitHub\FIRST-ROBOTICS-2018-5436-CAD\Field\FIRST Power Up Field CAD\Body_743_sldprt.ipt
- C:\Users\CAD\Documents\GitHub\FIRST-ROBOTICS-2018-5436-CAD\Field\FIRST Power Up Field CAD\Body_744_sldprt.ipt
- C:\Users\CAD\Documents\GitHub\FIRST-ROBOTICS-2018-5436-CAD\Field\FIRST Power Up Field CAD\Body_745_sldprt.ipt
- C:\Users\CAD\Documents\GitHub\FIRST-ROBOTICS-2018-5436-CAD\Field\FIRST Power Up Field CAD\Body_746_sldprt.ipt
- C:\Users\CAD\Documents\GitHub\FIRST-ROBOTICS-2018-5436-CAD\Field\FIRST Power Up Field CAD\Body_747_sldprt.ipt
- C:\Users\CAD\Documents\GitHub\FIRST-ROBOTICS-2018-5436-CAD\Field\FIRST Power Up Field CAD\Body_748_sldprt.ipt
- C:\Users\CAD\Documents\GitHub\FIRST-ROBOTICS-2018-5436-CAD\Field\FIRST Power Up Field CAD\Body_749_sldprt.ipt
- C:\Users\CAD\Documents\GitHub\FIRST-ROBOTICS-2018-5436-CAD\Field\FIRST Power Up Field CAD\Body_750_sldprt.ipt
- C:\Users\CAD\Documents\GitHub\FIRST-ROBOTICS-2018-5436-CAD\Field\FIRST Power Up Field CAD\Body_751_sldprt.ipt
- C:\Users\CAD\Documents\GitHub\FIRST-ROBOTICS-2018-5436-CAD\Field\FIRST Power Up Field CAD\Body_752_sldprt.ipt
- C:\Users\CAD\Documents\GitHub\FIRST-ROBOTICS-2018-5436-CAD\Field\FIRST Power Up Field CAD\Body_753_sldprt.ipt
- C:\Users\CAD\Documents\GitHub\FIRST-ROBOTICS-2018-5436-CAD\Field\FIRST Power Up Field CAD\Body_754_sldprt.ipt
- C:\Users\CAD\Documents\GitHub\FIRST-ROBOTICS-2018-5436-CAD\Field\FIRST Power Up Field CAD\Body_755_sldprt.ipt
- C:\Users\CAD\Documents\GitHub\FIRST-ROBOTICS-2018-5436-CAD\Field\FIRST Power Up Field CAD\Body_756_sldprt.ipt
- C:\Users\CAD\Documents\GitHub\FIRST-ROBOTICS-2018-5436-CAD\Field\FIRST Power Up Field CAD\Body_757_sldprt.ipt
- C:\Users\CAD\Documents\GitHub\FIRST-ROBOTICS-2018-5436-CAD\Field\FIRST Power Up Field CAD\Body_758_sldprt.ipt
- C:\Users\CAD\Documents\GitHub\FIRST-ROBOTICS-2018-5436-CAD\Field\FIRST Power Up Field CAD\Body_759_sldprt.ipt
- C:\Users\CAD\Documents\GitHub\FIRST-ROBOTICS-2018-5436-CAD\Field\FIRST Power Up Field CAD\Body_760_sldprt.ipt
- C:\Users\CAD\Documents\GitHub\FIRST-ROBOTICS-2018-5436-CAD\Field\FIRST Power Up Field CAD\Body_761_sldprt.ipt
- C:\Users\CAD\Documents\GitHub\FIRST-ROBOTICS-2018-5436-CAD\Field\FIRST Power Up Field CAD\Body_762_sldprt.ipt
- C:\Users\CAD\Documents\GitHub\FIRST-ROBOTICS-2018-5436-CAD\Field\FIRST Power Up Field CAD\Body_763_sldprt.ipt
- C:\Users\CAD\Documents\GitHub\FIRST-ROBOTICS-2018-5436-CAD\Field\FIRST Power Up Field CAD\Body_764_sldprt.ipt
- C:\Users\CAD\Documents\GitHub\FIRST-ROBOTICS-2018-5436-CAD\Field\FIRST Power Up Field CAD\Body_765_sldprt.ipt
- C:\Users\CAD\Documents\GitHub\FIRST-ROBOTICS-2018-5436-CAD\Field\FIRST Power Up Field CAD\Body_766_sldprt.ipt
- C:\Users\CAD\Documents\GitHub\FIRST-ROBOTICS-2018-5436-CAD\Field\FIRST Power Up Field CAD\Body_767_sldprt.ipt
- C:\Users\CAD\Documents\GitHub\FIRST-ROBOTICS-2018-5436-CAD\Field\FIRST Power Up Field CAD\Body_768_sldprt.ipt
- C:\Users\CAD\Documents\GitHub\FIRST-ROBOTICS-2018-5436-CAD\Field\FIRST Power Up Field CAD\Body_769_sldprt.ipt
- C:\Users\CAD\Documents\GitHub\FIRST-ROBOTICS-2018-5436-CAD\Field\FIRST Power Up Field CAD\Body_770_sldprt.ipt
- C:\Users\CAD\Documents\GitHub\FIRST-ROBOTICS-2018-5436-CAD\Field\FIRST Power Up Field CAD\Body_771_sldprt.ipt
- C:\Users\CAD\Documents\GitHub\FIRST-ROBOTICS-2018-5436-CAD\Field\FIRST Power Up Field CAD\Body_772_sldprt.ipt
- C:\Users\CAD\Documents\GitHub\FIRST-ROBOTICS-2018-5436-CAD\Field\FIRST Power Up Field CAD\Body_773_sldprt.ipt
- C:\Users\CAD\Documents\GitHub\FIRST-ROBOTICS-2018-5436-CAD\Field\FIRST Power Up Field CAD\Body_774_sldprt.ipt
- C:\Users\CAD\Documents\GitHub\FIRST-ROBOTICS-2018-5436-CAD\Field\FIRST Power Up Field CAD\Body_775_sldprt.ipt
- C:\Users\CAD\Documents\GitHub\FIRST-ROBOTICS-2018-5436-CAD\Field\FIRST Power Up Field CAD\Body_776_sldprt.ipt
- C:\Users\CAD\Documents\GitHub\FIRST-ROBOTICS-2018-5436-CAD\Field\FIRST Power Up Field CAD\Body_777_sldprt.ipt
- C:\Users\CAD\Documents\GitHub\FIRST-ROBOTICS-2018-5436-CAD\Field\FIRST Power Up Field CAD\Body_778_sldprt.ipt
- C:\Users\CAD\Documents\GitHub\FIRST-ROBOTICS-2018-5436-CAD\Field\FIRST Power Up Field CAD\Body_779_sldprt.ipt
- C:\Users\CAD\Documents\GitHub\FIRST-ROBOTICS-2018-5436-CAD\Field\FIRST Power Up Field CAD\Body_780_sldprt.ipt
- C:\Users\CAD\Documents\GitHub\FIRST-ROBOTICS-2018-5436-CAD\Field\FIRST Power Up Field CAD\Body_781_sldprt.ipt
- C:\Users\CAD\Documents\GitHub\FIRST-ROBOTICS-2018-5436-CAD\Field\FIRST Power Up Field CAD\Body_782_sldprt.ipt
- C:\Users\CAD\Documents\GitHub\FIRST-ROBOTICS-2018-5436-CAD\Field\FIRST Power Up Field CAD\Body_783_sldprt.ipt
- C:\Users\CAD\Documents\GitHub\FIRST-ROBOTICS-2018-5436-CAD\Field\FIRST Power Up Field CAD\Body_784_sldprt.ipt
- C:\Users\CAD\Documents\GitHub\FIRST-ROBOTICS-2018-5436-CAD\Field\FIRST Power Up Field CAD\Body_785_sldprt.ipt
- C:\Users\CAD\Documents\GitHub\FIRST-ROBOTICS-2018-5436-CAD\Field\FIRST Power Up Field CAD\Body_786_sldprt.ipt
- C:\Users\CAD\Documents\GitHub\FIRST-ROBOTICS-2018-5436-CAD\Field\FIRST Power Up Field CAD\Body_787_sldprt.ipt
- C:\Users\CAD\Documents\GitHub\FIRST-ROBOTICS-2018-5436-CAD\Field\FIRST Power Up Field CAD\Body_788_sldprt.ipt
- C:\Users\CAD\Documents\GitHub\FIRST-ROBOTICS-2018-5436-CAD\Field\FIRST Power Up Field CAD\Body_789_sldprt.ipt
- C:\Users\CAD\Documents\GitHub\FIRST-ROBOTICS-2018-5436-CAD\Field\FIRST Power Up Field CAD\Body_790_sldprt.ipt
- C:\Users\CAD\Documents\GitHub\FIRST-ROBOTICS-2018-5436-CAD\Field\FIRST Power Up Field CAD\Body_791_sldprt.ipt
- C:\Users\CAD\Documents\GitHub\FIRST-ROBOTICS-2018-5436-CAD\Field\FIRST Power Up Field CAD\Body_792_sldprt.ipt
- C:\Users\CAD\Documents\GitHub\FIRST-ROBOTICS-2018-5436-CAD\Field\FIRST Power Up Field CAD\Body_793_sldprt.ipt
- C:\Users\CAD\Documents\GitHub\FIRST-ROBOTICS-2018-5436-CAD\Field\FIRST Power Up Field CAD\Body_794_sldprt.ipt
- C:\Users\CAD\Documents\GitHub\FIRST-ROBOTICS-2018-5436-CAD\Field\FIRST Power Up Field CAD\Body_795_sldprt.ipt
- C:\Users\CAD\Documents\GitHub\FIRST-ROBOTICS-2018-5436-CAD\Field\FIRST Power Up Field CAD\Body_796_sldprt.ipt
- C:\Users\CAD\Documents\GitHub\FIRST-ROBOTICS-2018-5436-CAD\Field\FIRST Power Up Field CAD\Body_797_sldprt.ipt
- C:\Users\CAD\Documents\GitHub\FIRST-ROBOTICS-2018-5436-CAD\Field\FIRST Power Up Field CAD\Body_798_sldprt.ipt
- C:\Users\CAD\Documents\GitHub\FIRST-ROBOTICS-2018-5436-CAD\Field\FIRST Power Up Field CAD\Body_799_sldprt.ipt
- C:\Users\CAD\Documents\GitHub\FIRST-ROBOTICS-2018-5436-CAD\Field\FIRST Power Up Field CAD\Body_800_sldprt.ipt
- C:\Users\CAD\Documents\GitHub\FIRST-ROBOTICS-2018-5436-CAD\Field\FIRST Power Up Field CAD\Body_801_sldprt.ipt
- C:\Users\CAD\Documents\GitHub\FIRST-ROBOTICS-2018-5436-CAD\Field\FIRST Power Up Field CAD\Body_802_sldprt.ipt
- C:\Users\CAD\Documents\GitHub\FIRST-ROBOTICS-2018-5436-CAD\Field\FIRST Power Up Field CAD\Body_803_sldprt.ipt
- C:\Users\CAD\Documents\GitHub\FIRST-ROBOTICS-2018-5436-CAD\Field\FIRST Power Up Field CAD\Body_804_sldprt.ipt
- C:\Users\CAD\Documents\GitHub\FIRST-ROBOTICS-2018-5436-CAD\Field\FIRST Power Up Field CAD\Body_805_sldprt.ipt
- C:\Users\CAD\Documents\GitHub\FIRST-ROBOTICS-2018-5436-CAD\Field\FIRST Power Up Field CAD\Body_806_sldprt.ipt
- C:\Users\CAD\Documents\GitHub\FIRST-ROBOTICS-2018-5436-CAD\Field\FIRST Power Up Field CAD\Body_807_sldprt.ipt
- C:\Users\CAD\Documents\GitHub\FIRST-ROBOTICS-2018-5436-CAD\Field\FIRST Power Up Field CAD\Body_808_sldprt.ipt
- C:\Users\CAD\Documents\GitHub\FIRST-ROBOTICS-2018-5436-CAD\Field\FIRST Power Up Field CAD\Body_809_sldprt.ipt
- C:\Users\CAD\Documents\GitHub\FIRST-ROBOTICS-2018-5436-CAD\Field\FIRST Power Up Field CAD\Body_810_sldprt.ipt
- C:\Users\CAD\Documents\GitHub\FIRST-ROBOTICS-2018-5436-CAD\Field\FIRST Power Up Field CAD\Body_811_sldprt.ipt
- C:\Users\CAD\Documents\GitHub\FIRST-ROBOTICS-2018-5436-CAD\Field\FIRST Power Up Field CAD\Body_812_sldprt.ipt
- C:\Users\CAD\Documents\GitHub\FIRST-ROBOTICS-2018-5436-CAD\Field\FIRST Power Up Field CAD\Body_813_sldprt.ipt
- C:\Users\CAD\Documents\GitHub\FIRST-ROBOTICS-2018-5436-CAD\Field\FIRST Power Up Field CAD\Body_814_sldprt.ipt
- C:\Users\CAD\Documents\GitHub\FIRST-ROBOTICS-2018-5436-CAD\Field\FIRST Power Up Field CAD\Body_815_sldprt.ipt
- C:\Users\CAD\Documents\GitHub\FIRST-ROBOTICS-2018-5436-CAD\Field\FIRST Power Up Field CAD\Body_816_sldprt.ipt
- C:\Users\CAD\Documents\GitHub\FIRST-ROBOTICS-2018-5436-CAD\Field\FIRST Power Up Field CAD\Body_817_sldprt.ipt
- C:\Users\CAD\Documents\GitHub\FIRST-ROBOTICS-2018-5436-CAD\Field\FIRST Power Up Field CAD\Body_818_sldprt.ipt
- C:\Users\CAD\Documents\GitHub\FIRST-ROBOTICS-2018-5436-CAD\Field\FIRST Power Up Field CAD\Body_819_sldprt.ipt
- C:\Users\CAD\Documents\GitHub\FIRST-ROBOTICS-2018-5436-CAD\Field\FIRST Power Up Field CAD\Body_820_sldprt.ipt
- C:\Users\CAD\Documents\GitHub\FIRST-ROBOTICS-2018-5436-CAD\Field\FIRST Power Up Field CAD\Body_821_sldprt.ipt
- C:\Users\CAD\Documents\GitHub\FIRST-ROBOTICS-2018-5436-CAD\Field\FIRST Power Up Field CAD\Body_822_sldprt.ipt
- C:\Users\CAD\Documents\GitHub\FIRST-ROBOTICS-2018-5436-CAD\Field\FIRST Power Up Field CAD\Body_823_sldprt.ipt
- C:\Users\CAD\Documents\GitHub\FIRST-ROBOTICS-2018-5436-CAD\Field\FIRST Power Up Field CAD\Body_824_sldprt.ipt
- C:\Users\CAD\Documents\GitHub\FIRST-ROBOTICS-2018-5436-CAD\Field\FIRST Power Up Field CAD\Body_825_sldprt.ipt
- C:\Users\CAD\Documents\GitHub\FIRST-ROBOTICS-2018-5436-CAD\Field\FIRST Power Up Field CAD\Body_826_sldprt.ipt
- C:\Users\CAD\Documents\GitHub\FIRST-ROBOTICS-2018-5436-CAD\Field\FIRST Power Up Field CAD\Body_827_sldprt.ipt
- C:\Users\CAD\Documents\GitHub\FIRST-ROBOTICS-2018-5436-CAD\Field\FIRST Power Up Field CAD\Body_828_sldprt.ipt
- C:\Users\CAD\Documents\GitHub\FIRST-ROBOTICS-2018-5436-CAD\Field\FIRST Power Up Field CAD\Body_829_sldprt.ipt
- C:\Users\CAD\Documents\GitHub\FIRST-ROBOTICS-2018-5436-CAD\Field\FIRST Power Up Field CAD\Body_830_sldprt.ipt
- C:\Users\CAD\Documents\GitHub\FIRST-ROBOTICS-2018-5436-CAD\Field\FIRST Power Up Field CAD\Body_831_sldprt.ipt
- C:\Users\CAD\Documents\GitHub\FIRST-ROBOTICS-2018-5436-CAD\Field\FIRST Power Up Field CAD\Body_832_sldprt.ipt
- C:\Users\CAD\Documents\GitHub\FIRST-ROBOTICS-2018-5436-CAD\Field\FIRST Power Up Field CAD\Body_833_sldprt.ipt
- C:\Users\CAD\Documents\GitHub\FIRST-ROBOTICS-2018-5436-CAD\Field\FIRST Power Up Field CAD\Body_834_sldprt.ipt
- C:\Users\CAD\Documents\GitHub\FIRST-ROBOTICS-2018-5436-CAD\Field\FIRST Power Up Field CAD\Body_835_sldprt.ipt
- C:\Users\CAD\Documents\GitHub\FIRST-ROBOTICS-2018-5436-CAD\Field\FIRST Power Up Field CAD\Body_836_sldprt.ipt
- C:\Users\CAD\Documents\GitHub\FIRST-ROBOTICS-2018-5436-CAD\Field\FIRST Power Up Field CAD\Body_837_sldprt.ipt
- C:\Users\CAD\Documents\GitHub\FIRST-ROBOTICS-2018-5436-CAD\Field\FIRST Power Up Field CAD\Body_838_sldprt.ipt
- C:\Users\CAD\Documents\GitHub\FIRST-ROBOTICS-2018-5436-CAD\Field\FIRST Power Up Field CAD\Body_839_sldprt.ipt
- C:\Users\CAD\Documents\GitHub\FIRST-ROBOTICS-2018-5436-CAD\Field\FIRST Power Up Field CAD\Body_840_sldprt.ipt
- C:\Users\CAD\Documents\GitHub\FIRST-ROBOTICS-2018-5436-CAD\Field\FIRST Power Up Field CAD\Body_841_sldprt.ipt
- C:\Users\CAD\Documents\GitHub\FIRST-ROBOTICS-2018-5436-CAD\Field\FIRST Power Up Field CAD\Body_842_sldprt.ipt
- C:\Users\CAD\Documents\GitHub\FIRST-ROBOTICS-2018-5436-CAD\Field\FIRST Power Up Field CAD\Body_843_sldprt.ipt
- C:\Users\CAD\Documents\GitHub\FIRST-ROBOTICS-2018-5436-CAD\Field\FIRST Power Up Field CAD\Body_844_sldprt.ipt
- C:\Users\CAD\Documents\GitHub\FIRST-ROBOTICS-2018-5436-CAD\Field\FIRST Power Up Field CAD\Body_845_sldprt.ipt
- C:\Users\CAD\Documents\GitHub\FIRST-ROBOTICS-2018-5436-CAD\Field\FIRST Power Up Field CAD\Body_846_sldprt.ipt
- C:\Users\CAD\Documents\GitHub\FIRST-ROBOTICS-2018-5436-CAD\Field\FIRST Power Up Field CAD\Body_847_sldprt.ipt
- C:\Users\CAD\Documents\GitHub\FIRST-ROBOTICS-2018-5436-CAD\Field\FIRST Power Up Field CAD\Body_848_sldprt.ipt
- C:\Users\CAD\Documents\GitHub\FIRST-ROBOTICS-2018-5436-CAD\Field\FIRST Power Up Field CAD\Body_849_sldprt.ipt
- C:\Users\CAD\Documents\GitHub\FIRST-ROBOTICS-2018-5436-CAD\Field\FIRST Power Up Field CAD\Body_850_sldprt.ipt
- C:\Users\CAD\Documents\GitHub\FIRST-ROBOTICS-2018-5436-CAD\Field\FIRST Power Up Field CAD\Body_851_sldprt.ipt
- C:\Users\CAD\Documents\GitHub\FIRST-ROBOTICS-2018-5436-CAD\Field\FIRST Power Up Field CAD\Body_852_sldprt.ipt
- C:\Users\CAD\Documents\GitHub\FIRST-ROBOTICS-2018-5436-CAD\Field\FIRST Power Up Field CAD\Body_853_sldprt.ipt
- C:\Users\CAD\Documents\GitHub\FIRST-ROBOTICS-2018-5436-CAD\Field\FIRST Power Up Field CAD\Body_854_sldprt.ipt
- C:\Users\CAD\Documents\GitHub\FIRST-ROBOTICS-2018-5436-CAD\Field\FIRST Power Up Field CAD\Body_855_sldprt.ipt
- C:\Users\CAD\Documents\GitHub\FIRST-ROBOTICS-2018-5436-CAD\Field\FIRST Power Up Field CAD\Body_856_sldprt.ipt
- C:\Users\CAD\Documents\GitHub\FIRST-ROBOTICS-2018-5436-CAD\Field\FIRST Power Up Field CAD\Body_857_sldprt.ipt